# Autodesk Inventor assembly: LED组装
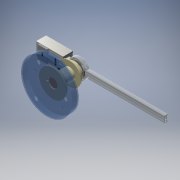
[picture p0: Inventor's stored thumbnail of the model, 180x180]
Saved by Autodesk Inventor 2018 (Build 220112000, 112)
## iProperties
Created: 2020-11-22
Part Number: LED组装
Material: 常规
Document SubType Name: Assembly
Designer: OHHHHHHHHHH
Author: OHHHHHHHHHH
## Documents named in this file (15)
- F:\大三上学习记录\电工开放性实验：LED阵列显示\3D建模\LED组装.iam
- F:\大三上学习记录\电工开放性实验：LED阵列显示\3D建模\底盘.ipt
- F:\大三上学习记录\电工开放性实验：LED阵列显示\3D建模\电机帽.ipt
- F:\大三上学习记录\电工开放性实验：LED阵列显示\3D建模\转动部分.ipt
- F:\大三上学习记录\电工开放性实验：LED阵列显示\3D建模\电机.ipt
- F:\大三上学习记录\电工开放性实验：LED阵列显示\3D建模\线圈.ipt
- F:\大三上学习记录\电工开放性实验：LED阵列显示\3D建模\装置容器.ipt
- F:\大三上学习记录\电工开放性实验：LED阵列显示\3D建模\无线发射模块.ipt
- F:\大三上学习记录\电工开放性实验：LED阵列显示\3D建模\无线接收模块.ipt
- F:\大三上学习记录\电工开放性实验：LED阵列显示\3D建模\51单片机.ipt
- F:\大三上学习记录\电工开放性实验：LED阵列显示\3D建模\洞洞板.ipt
- F:\大三上学习记录\电工开放性实验：LED阵列显示\3D建模\稳压.ipt
- F:\大三上学习记录\电工开放性实验：LED阵列显示\3D建模\battery.ipt
- F:\大三上学习记录\电工开放性实验：LED阵列显示\3D建模\锁销.ipt
- F:\大三上学习记录\电工开放性实验：LED阵列显示\3D建模\盖板.ipt
## Components (15 placed, 14 different names)
1. 底盘:1 — 配合:1, 配合:26
2. 电机帽:1 — 配合:1, 配合:3, 配合:4, 表面齐平:1, 配合:7, 配合:8, 配合:17, 配合:18, 表面齐平:9, 配合:19, 表面齐平:10, 配合:20, 配合:21, 配合:26
3. 转动部分:1 — 配合:3, 配合:5, 配合:6, 角度:1, 配合:10, 配合:11, 表面齐平:2, 配合:22, 配合:23, 角度:2
4. 电机:1 — 配合:4, 表面齐平:1, 角度:1
5. 线圈:1 — 配合:5, 配合:6, 配合:9
6. 线圈:2 — 配合:7, 配合:8, 配合:9
7. 装置容器:1 — 配合:10, 配合:11, 表面齐平:2, 配合:12, 表面齐平:3, 配合:14, 表面齐平:6, 配合:15, 表面齐平:7, 表面齐平:8, 配合:24, 配合:25
8. 无线发射模块:1 — 配合:17, 配合:18, 表面齐平:9
9. 无线接收模块:1 — 配合:12, 表面齐平:3, 配合:16
10. 51单片机:1 — 配合:13, 表面齐平:4, 表面齐平:5
11. 洞洞板:1 — 配合:13, 表面齐平:4, 表面齐平:5, 配合:14, 表面齐平:6
12. 稳压:1 — 配合:15, 表面齐平:7, 配合:16, 表面齐平:8
13. battery:1 — 配合:19, 表面齐平:10, 配合:20, 配合:21
14. 锁销:1 — 配合:22, 配合:23, 角度:2
15. 盖板:1 — 配合:24, 配合:25
## Relationships (37: Mate 25, Flush 10, Angle 2)
- 配合:1 [Mate]: 底盘:1 ↔ 电机帽:1
- 配合:3 [Mate]: 电机帽:1 ↔ 转动部分:1
- 配合:4 [Mate]: 电机帽:1 ↔ 电机:1
- 表面齐平:1 [Flush]: 电机帽:1 ↔ 电机:1
- 配合:5 [Mate]: 转动部分:1 ↔ 线圈:1
- 配合:6 [Mate]: 转动部分:1 ↔ 线圈:1
- 配合:7 [Mate]: 电机帽:1 ↔ 线圈:2
- 配合:8 [Mate]: 电机帽:1 ↔ 线圈:2
- 角度:1 [Angle] (0 deg): 转动部分:1 ↔ 电机:1
- 配合:9 [Mate] (3 mm): 线圈:1 ↔ 线圈:2
- 配合:10 [Mate]: 转动部分:1 ↔ 装置容器:1
- 配合:11 [Mate]: 转动部分:1 ↔ 装置容器:1
- 表面齐平:2 [Flush]: 转动部分:1 ↔ 装置容器:1
- 配合:12 [Mate]: 装置容器:1 ↔ 无线接收模块:1
- 表面齐平:3 [Flush] (9 mm): 装置容器:1 ↔ 无线接收模块:1
- 配合:13 [Mate]: 51单片机:1 ↔ 洞洞板:1
- 表面齐平:4 [Flush]: 51单片机:1 ↔ 洞洞板:1
- 表面齐平:5 [Flush] (-3 mm): 51单片机:1 ↔ 洞洞板:1
- 配合:14 [Mate] (15 mm): 装置容器:1 ↔ 洞洞板:1
- 表面齐平:6 [Flush] (5 mm): 装置容器:1 ↔ 洞洞板:1
- 配合:15 [Mate]: 装置容器:1 ↔ 稳压:1
- 表面齐平:7 [Flush] (-0.5 mm): 装置容器:1 ↔ 稳压:1
- 配合:16 [Mate] (3.5 mm): 无线接收模块:1 ↔ 稳压:1
- 表面齐平:8 [Flush] (9 mm): 装置容器:1 ↔ 稳压:1
- 配合:17 [Mate]: 电机帽:1 ↔ 无线发射模块:1
- 配合:18 [Mate]: 电机帽:1 ↔ 无线发射模块:1
- 表面齐平:9 [Flush] (-8.5 mm): 电机帽:1 ↔ 无线发射模块:1
- 配合:19 [Mate]: 电机帽:1 ↔ battery:1
- 表面齐平:10 [Flush] (2.5 mm): 电机帽:1 ↔ battery:1
- 配合:20 [Mate]: 电机帽:1 ↔ battery:1
- 配合:21 [Mate] (0.5 mm): 电机帽:1 ↔ battery:1
- 配合:22 [Mate]: 转动部分:1 ↔ 锁销:1
- 配合:23 [Mate]: 转动部分:1 ↔ 锁销:1
- 角度:2 [Angle] (0 deg): 转动部分:1 ↔ 锁销:1
- 配合:24 [Mate]: 装置容器:1 ↔ 盖板:1
- 配合:25 [Mate]: 装置容器:1 ↔ 盖板:1
- 配合:26 [Mate]: 底盘:1 ↔ 电机帽:1
